# Autodesk Inventor assembly: 1x2 Angle
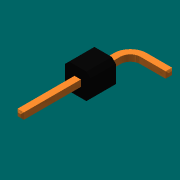
[picture p0: Inventor's stored thumbnail of the model, 180x180]
Saved by Autodesk Inventor 2016 SP1 (Build 200210100, 210)
## iProperties
Created: 2014-10-18
Part Number: 1x2 Angle
Document SubType Name: Assembly
Designer: Sawaiz Syed
Author: Sawaiz Syed
## Documents named in this file (3)
- C:\Users\sawai\OneDrive\projects\mppcInterface\cad\connector\2.54Header\rightAngle\1x1Angle.iam
- C:\Users\sawai\OneDrive\projects\mppcInterface\cad\connector\2.54Header\rightAngle\Holder.ipt
- C:\Users\sawai\OneDrive\projects\mppcInterface\cad\connector\2.54Header\rightAngle\PinRight.ipt
## Components (2 placed, 2 different names)
1. Holder:2 — Mate:4, Mate:5, Flush:1
2. PinRight:1 — Mate:4, Mate:5, Flush:1
## Relationships (3: Mate 2, Flush 1)
- Mate:4: Holder:2 ↔ PinRight:1
- Mate:5: Holder:2 ↔ PinRight:1
- Flush:1 (-5.84 mm): Holder:2 ↔ PinRight:1
